# Autodesk Inventor assembly: PlanetaryGearbox
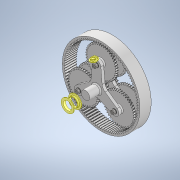
[picture p0: Inventor's stored thumbnail of the model, 180x180]
Saved by Autodesk Inventor 2020 (Build 240168000, 168)
## iProperties
Created: 2020-05-11
Part Number: PlanetaryGearbox
Document SubType Name: Assembly
Designer: avi41
Author: avi41
## Documents named in this file (12)
- C:\Users\avi41\Desktop\CAD Robot Arm\PlanetaryGearbox.iam
- C:\Users\avi41\Desktop\CAD Robot Arm\Ring_gear.ipt
- C:\Users\avi41\Desktop\CAD Robot Arm\Stage1_sun_gear.ipt
- C:\Users\avi41\Desktop\CAD Robot Arm\Stage1_planet_gear.ipt
- C:\Users\avi41\Desktop\CAD Robot Arm\Stage2_sun_gear.ipt
- C:\Users\avi41\Desktop\CAD Robot Arm\Stage2_planet_gear.ipt
- C:\Users\avi41\Desktop\CAD Robot Arm\Shaft_interstage.ipt
- C:\Users\avi41\Documents\Inventor\Content Center Files\R2020\en-US\ISO 8738(1)\ISO 8738 - 4(1).ipt
- C:\Users\avi41\Desktop\CAD Robot Arm\Shaft_output.ipt
- C:\Users\avi41\Documents\Inventor\Content Center Files\R2020\en-US\DIN 912\DIN 912 - M4 x 0.7 x 12 x 10.25.ipt
- C:\Users\avi41\Desktop\CAD Robot Arm\JFM_1517_04_2.ipt
- C:\Users\avi41\Desktop\CAD Robot Arm\JFM_0507_03_1.ipt
## Components (27 placed, 11 different names)
1. Ring_gear:1 — Mate:1, Mate:2, Flush:1, Mate:3, Flush:2, Flush:9, Flush:10, Flush:11, Flush:12, Flush:13
2. Stage1_sun_gear:1 — Mate:3, Flush:2, Mate:10, Flush:10
3. Stage1_planet_gear:1 — Mate:6, Flush:11, Mate:11, Mate:16
4. Stage1_planet_gear:2 — Mate:5, Flush:13, Mate:12, Mate:14
5. Stage1_planet_gear:3 — Mate:4, Flush:12, Mate:13
6. Stage2_sun_gear:1 — Flush:9, Mate:10, Flush:14, Flush:15, Flush:16, Mate:15
7. Stage2_planet_gear:1 — Flush:15, Mate:13, Mate:29
8. Stage2_planet_gear:2 — Flush:14, Mate:11, Mate:30
9. Stage2_planet_gear:3 — Flush:16, Mate:12
10. Shaft_interstage:1 — Mate:14, Mate:15, Mate:16, Mate:23, Mate:24, Mate:25, Mate:26, Mate:27, Mate:28, Mate:31
11. Shaft_output:1 — Mate:29, Mate:30, Mate:31, Mate:38, Mate:39, Mate:40, Mate:41, Mate:42, Mate:43, Mate:44, Mate:45
12. JFM_1517_04_2:1 — Mate:44
13. JFM_1517_04_2:2 — Mate:45
14. JFM_0507_03_1:1
15. JFM_0507_03_1:2
16. DIN 912 - replaced by DIN EN ISO 4762 M4 x 12:1 — Mate:17, Mate:18, Mate:26
17. DIN 912 - replaced by DIN EN ISO 4762 M4 x 12:2 — Mate:19, Mate:20, Mate:28
18. DIN 912 - replaced by DIN EN ISO 4762 M4 x 12:3 — Mate:21, Mate:22, Mate:27
19. DIN EN 28738 4:1 — Mate:17, Mate:18, Mate:25
20. DIN EN 28738 4:2 — Mate:19, Mate:20, Mate:24
21. DIN EN 28738 4:3 — Mate:21, Mate:22, Mate:23
22. DIN EN 28738 4:4 — Mate:32, Mate:36, Mate:42
23. DIN EN 28738 4:5 — Mate:34, Mate:35, Mate:41
24. DIN EN 28738 4:6 — Mate:33, Mate:37, Mate:43
25. DIN 912 - replaced by DIN EN ISO 4762 M4 x 12:4 — Mate:33, Mate:37, Mate:38
26. DIN 912 - replaced by DIN EN ISO 4762 M4 x 12:5 — Mate:34, Mate:35, Mate:40
27. DIN 912 - replaced by DIN EN ISO 4762 M4 x 12:6 — Mate:32, Mate:36, Mate:39
## Relationships (52: Mate 42, Flush 10)
- Mate:1: Ring_gear:1
- Mate:2: Ring_gear:1
- Flush:1: Ring_gear:1
- Mate:3: Ring_gear:1 ↔ Stage1_sun_gear:1
- Flush:2: Ring_gear:1 ↔ Stage1_sun_gear:1
- Mate:4: Stage1_planet_gear:3
- Mate:5: Stage1_planet_gear:2
- Mate:6: Stage1_planet_gear:1
- Flush:9: Ring_gear:1 ↔ Stage2_sun_gear:1
- Mate:10: Stage1_sun_gear:1 ↔ Stage2_sun_gear:1
- Flush:10: Ring_gear:1 ↔ Stage1_sun_gear:1
- Flush:11: Ring_gear:1 ↔ Stage1_planet_gear:1
- Flush:12: Ring_gear:1 ↔ Stage1_planet_gear:3
- Flush:13: Ring_gear:1 ↔ Stage1_planet_gear:2
- Flush:14: Stage2_sun_gear:1 ↔ Stage2_planet_gear:2
- Flush:15: Stage2_sun_gear:1 ↔ Stage2_planet_gear:1
- Flush:16: Stage2_sun_gear:1 ↔ Stage2_planet_gear:3
- Mate:11: Stage1_planet_gear:1 ↔ Stage2_planet_gear:2
- Mate:12: Stage1_planet_gear:2 ↔ Stage2_planet_gear:3
- Mate:13: Stage1_planet_gear:3 ↔ Stage2_planet_gear:1
- Mate:14: Stage1_planet_gear:2 ↔ Shaft_interstage:1
- Mate:15: Stage2_sun_gear:1 ↔ Shaft_interstage:1
- Mate:16: Stage1_planet_gear:1 ↔ Shaft_interstage:1
- Mate:17: DIN 912 - replaced by DIN EN ISO 4762 M4 x 12:1 ↔ DIN EN 28738 4:1
- Mate:18: DIN 912 - replaced by DIN EN ISO 4762 M4 x 12:1 ↔ DIN EN 28738 4:1
- Mate:19: DIN 912 - replaced by DIN EN ISO 4762 M4 x 12:2 ↔ DIN EN 28738 4:2
- Mate:20: DIN 912 - replaced by DIN EN ISO 4762 M4 x 12:2 ↔ DIN EN 28738 4:2
- Mate:21: DIN 912 - replaced by DIN EN ISO 4762 M4 x 12:3 ↔ DIN EN 28738 4:3
- Mate:22: DIN 912 - replaced by DIN EN ISO 4762 M4 x 12:3 ↔ DIN EN 28738 4:3
- Mate:23: Shaft_interstage:1 ↔ DIN EN 28738 4:3
- Mate:24: Shaft_interstage:1 ↔ DIN EN 28738 4:2
- Mate:25: Shaft_interstage:1 ↔ DIN EN 28738 4:1
- Mate:26: Shaft_interstage:1 ↔ DIN 912 - replaced by DIN EN ISO 4762 M4 x 12:1
- Mate:27: Shaft_interstage:1 ↔ DIN 912 - replaced by DIN EN ISO 4762 M4 x 12:3
- Mate:28: Shaft_interstage:1 ↔ DIN 912 - replaced by DIN EN ISO 4762 M4 x 12:2
- Mate:29: Stage2_planet_gear:1 ↔ Shaft_output:1
- Mate:30: Stage2_planet_gear:2 ↔ Shaft_output:1
- Mate:31: Shaft_interstage:1 ↔ Shaft_output:1
- Mate:32: DIN EN 28738 4:4 ↔ DIN 912 - replaced by DIN EN ISO 4762 M4 x 12:6
- Mate:33: DIN EN 28738 4:6 ↔ DIN 912 - replaced by DIN EN ISO 4762 M4 x 12:4
- Mate:34: DIN EN 28738 4:5 ↔ DIN 912 - replaced by DIN EN ISO 4762 M4 x 12:5
- Mate:35: DIN EN 28738 4:5 ↔ DIN 912 - replaced by DIN EN ISO 4762 M4 x 12:5
- Mate:36: DIN EN 28738 4:4 ↔ DIN 912 - replaced by DIN EN ISO 4762 M4 x 12:6
- Mate:37: DIN EN 28738 4:6 ↔ DIN 912 - replaced by DIN EN ISO 4762 M4 x 12:4
- Mate:38: Shaft_output:1 ↔ DIN 912 - replaced by DIN EN ISO 4762 M4 x 12:4
- Mate:39: Shaft_output:1 ↔ DIN 912 - replaced by DIN EN ISO 4762 M4 x 12:6
- Mate:40: Shaft_output:1 ↔ DIN 912 - replaced by DIN EN ISO 4762 M4 x 12:5
- Mate:41: Shaft_output:1 ↔ DIN EN 28738 4:5
- Mate:42: Shaft_output:1 ↔ DIN EN 28738 4:4
- Mate:43: Shaft_output:1 ↔ DIN EN 28738 4:6
- Mate:44: Shaft_output:1 ↔ JFM_1517_04_2:1
- Mate:45: Shaft_output:1 ↔ JFM_1517_04_2:2
